# Autodesk Inventor assembly: Drive Assembly
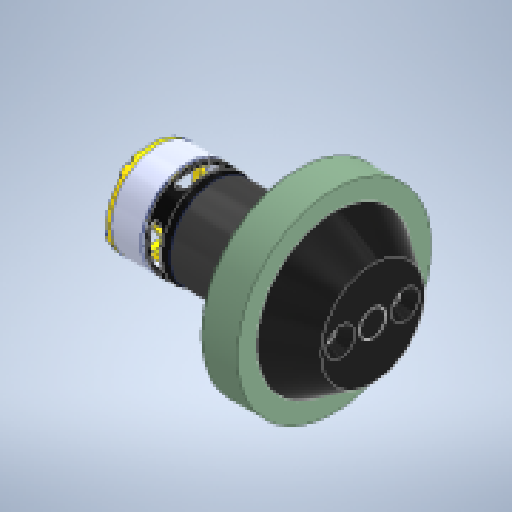
[picture p0: Inventor's stored thumbnail of the model, 512x512]
Saved by Autodesk Inventor 2023.2 (Build 272271000, 271)
## iProperties
Created: 2022-09-11
Part Number: Drive Assembly
Document SubType Name: Assembly
Designer: NCai2
Mass: 102.415 g
Surface Area: 201.007 cm^2
Volume: 29.1024 cm^3
Density: 3.51912 g/cm^3
Author: NCai2
## Documents named in this file (3)
- C:\Users\Nathan Cai\Documents\Inventor\Moon Cake V0.15\Drive Assembly.iam
- C:\Users\Nathan Cai\Documents\Inventor\Moon Cake V0.15\RR Brushless\RR-Brushless-Planetary.iam
- C:\Users\Nathan Cai\Documents\Inventor\Moon Cake V0.15\Custom Wheel V1.0\Recessed Wheels V1.0.iam
## Components (2 placed, 2 different names)
1. RR-Brushless-Planetary:1 [sub-assembly] — Mate:1, Mate:2
2. Recessed Wheels V1.0:1 [sub-assembly] — Mate:1, Mate:2
## Relationships (2: Mate 2)
- Mate:1 (-1 mm): RR-Brushless-Planetary:1 ↔ Recessed Wheels V1.0:1
- Mate:2: RR-Brushless-Planetary:1 ↔ Recessed Wheels V1.0:1
